# Autodesk Inventor assembly: Mech Motor_Wheel_BevelGears
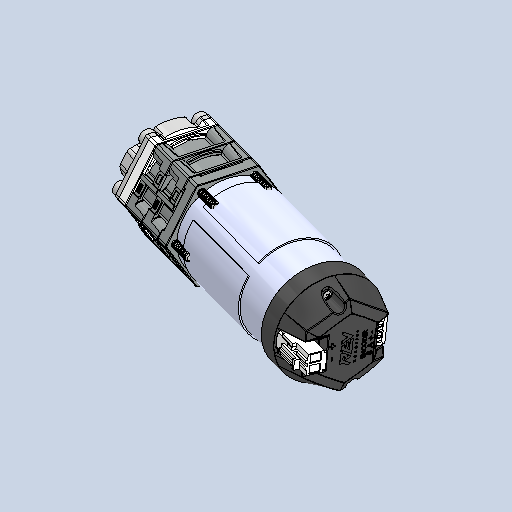
[picture p0: Inventor's stored thumbnail of the model, 512x512]
Saved by Autodesk Inventor 2023 (Build 270158000, 158)
## iProperties
Created: 2022-09-24
Part Number: Mech Motor_Wheel_BevelGears
Document SubType Name: Assembly
Designer: matt
Author: matt
## Documents named in this file (2)
- C:\Users\matt\Documents\Inventor\FTC\2022-23 FTC\Mech Chassis\Mech Motor_Wheel_BevelGears.iam
- C:\Users\matt\Documents\Inventor\FTC\2022-23 FTC\Motors\REV Ultraplanetary Motor 2 Cartridges.iam
## Components (1 placed, 1 different names)
1. REV Ultraplanetary Motor 2 Cartridges:1 [sub-assembly] — Angle:2
## Relationships (1: Angle 1)
- Angle:2 (0 deg): REV Ultraplanetary Motor 2 Cartridges:1
